# Autodesk Inventor assembly: ASY PNS 00 Panaevsk VOS
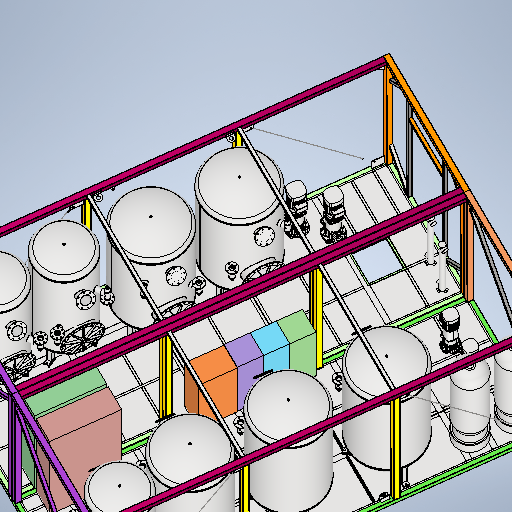
[picture p0: Inventor's stored thumbnail of the model, 512x512]
Saved by Autodesk Inventor 2025 (Build 290162010, 162A)
## iProperties
Created: 2025-02-24
Part Number: ASY PNS 00 Panaevsk VOS
Document SubType Name: Assembly
Designer: user
Author: user
## Documents named in this file (19)
- C:\Users\admin\Desktop\PNS-Panaevsk\ASY PNS 00 Panaevsk VOS.iam
- C:\Users\admin\Desktop\PNS-Panaevsk\Filter D1200\ASY PNS-Filter column D1200.iam
- C:\Users\admin\Desktop\PNS-Panaevsk\Filter D1000\ASY PNS-Filter column D1000.iam
- C:\Users\admin\Desktop\PNS-Panaevsk\ASY PNS-0100 MAIN FRAME.iam
- C:\Users\admin\Desktop\PNS-Panaevsk\ASY PNS-0200 FRAME 2.ipt
- C:\Users\admin\Desktop\PNS-Panaevsk\PNS-0921 concrete plate.ipt
- C:\Users\admin\Desktop\PNS-Panaevsk\PNS-0931 Sandwich wall.ipt
- C:\Users\admin\Desktop\PNS-Panaevsk\PNS-0932 Sandwich wall roof.ipt
- C:\Users\admin\Desktop\PNS-Panaevsk\PNS-0264 roof beam.ipt
- C:\Users\admin\Desktop\PNS-Panaevsk\Оборудование Инвентор\Вертикальный насос\CDM(F)15-4 FSWP(S_L)C\CDM(F)15-4 FSWP(S_L)C.iam
- C:\Users\admin\Desktop\PNS-Panaevsk\Оборудование Инвентор\Вертикальный насос\CDM(F)65-2-2 FSWP(S)C\CDM(F)65-2-2 FSWP(S)C.iam
- C:\Users\admin\Desktop\PNS-Panaevsk\Оборудование Инвентор\HY-H H2162–4T.ipt
- C:\Users\admin\Desktop\PNS-Panaevsk\Оборудование Инвентор\UV-Cleaner ODV-15.ipt
- C:\Users\admin\Desktop\PNS-Panaevsk\Оборудование Инвентор\Шкафы управления\Control box №1.ipt
- C:\Users\admin\Desktop\PNS-Panaevsk\Оборудование Инвентор\Шкафы управления\Control box №2.ipt
- C:\Users\admin\Desktop\PNS-Panaevsk\Оборудование Инвентор\Станции дозирования\Coagulant barrel.ipt
- C:\Users\admin\Desktop\PNS-Panaevsk\Оборудование Инвентор\Станции дозирования\Flocculant barrel.ipt
- C:\Users\admin\Desktop\PNS-Panaevsk\Оборудование Инвентор\Станции дозирования\GPHN barrel.ipt
- C:\Users\admin\Desktop\PNS-Panaevsk\Оборудование Инвентор\Станции дозирования\Soda barrel.ipt
## Components (34 placed, 18 different names)
1. ASY PNS-Filter column D1200:2 [sub-assembly] — Rigid:13
2. ASY PNS-Filter column D1000:3 [sub-assembly] — Rigid:16
3. ASY PNS-Filter column D1000:5 [sub-assembly] — Rigid:18
4. ASY PNS-0100 MAIN FRAME:1 [sub-assembly] — Rigid:1, Rigid:3, Rigid:4, Rigid:5, Rigid:7, Rigid:8, Rigid:9, Rigid:12, Rigid:13, Mate:15, Mate:16, Mate:17, Mate:18, Mate:19, Mate:20, Mate:21, Mate:22, Mate:23, Mate:24, Mate:26, Mate:27, Rigid:16, Rigid:17, Rigid:18
5. ASY PNS-0200 FRAME 2:1
6. ASY PNS-Filter column D1200:5 [sub-assembly] — Rigid:12
7. ASY PNS-Filter column D1200:6 [sub-assembly] — Rigid:8
8. ASY PNS-Filter column D1200:7 [sub-assembly] — Rigid:9
9. PNS-0931 Sandwich wall:1 — Rigid:1
10. PNS-0932 Sandwich wall roof:1 — Rigid:2
11. PNS-0932 Sandwich wall roof:2 — Rigid:2
12. PNS-0264 roof beam:1 — Rigid:3
13. PNS-0264 roof beam:2 — Rigid:4
14. PNS-0264 roof beam:3 — Rigid:5
15. ASY PNS-Filter column D1200:8 [sub-assembly] — Rigid:7
16. ASY PNS-Filter column D1000:6 [sub-assembly] — Rigid:17
17. CDM(F)15-4 FSWP(S_L)C:1 [sub-assembly] — Mate:16
18. CDM(F)65-2-2 FSWP(S)C:1 [sub-assembly] — Mate:18
19. HY-H H2162–4T:1 — Mate:19
20. UV-Cleaner ODV-15:1 — Mate:22
21. UV-Cleaner ODV-15:2 — Mate:21
22. HY-H H2162–4T:2 — Mate:20
23. CDM(F)65-2-2 FSWP(S)C:2 [sub-assembly] — Mate:17
24. CDM(F)15-4 FSWP(S_L)C:2 [sub-assembly] — Mate:15
25. Control box №1:1 — Mate:23, Mate:25, Flush:8
26. Control box №2:1 — Mate:24, Mate:25, Flush:8
27. Coagulant barrel:1 — Rigid:14, Rigid:15
28. Flocculant barrel:1 — Rigid:15, Mate:26
29. GPHN barrel:1 — Mate:27
30. Soda barrel:1 — Rigid:14
31. PNS-0921 concrete plate:1 — Flush:6, Flush:7, Mate:14
32. PNS-0921 concrete plate:2
33. PNS-0921 concrete plate:3
34. PNS-0921 concrete plate:4
## Component patterns: (4 elements, first: PNS-0921 concrete plate:1)
## Relationships (32: WeldJoint 15, Mate 14, Flush 3)
- Flush:6: PNS-0921 concrete plate:1
- Flush:7: PNS-0921 concrete plate:1
- Mate:14 (-500 mm): PNS-0921 concrete plate:1
- Rigid:1 [WeldJoint]: ASY PNS-0100 MAIN FRAME:1 ↔ PNS-0931 Sandwich wall:1
- Rigid:2 [WeldJoint]: PNS-0932 Sandwich wall roof:1 ↔ PNS-0932 Sandwich wall roof:2
- Rigid:3 [WeldJoint]: ASY PNS-0100 MAIN FRAME:1 ↔ PNS-0264 roof beam:1
- Rigid:4 [WeldJoint]: ASY PNS-0100 MAIN FRAME:1 ↔ PNS-0264 roof beam:2
- Rigid:5 [WeldJoint]: ASY PNS-0100 MAIN FRAME:1 ↔ PNS-0264 roof beam:3
- Rigid:7 [WeldJoint] (40 mm): ASY PNS-0100 MAIN FRAME:1 ↔ ASY PNS-Filter column D1200:8
- Rigid:8 [WeldJoint] (40 mm): ASY PNS-0100 MAIN FRAME:1 ↔ ASY PNS-Filter column D1200:6
- Rigid:9 [WeldJoint] (40 mm): ASY PNS-0100 MAIN FRAME:1 ↔ ASY PNS-Filter column D1200:7
- Rigid:12 [WeldJoint] (40 mm): ASY PNS-0100 MAIN FRAME:1 ↔ ASY PNS-Filter column D1200:5
- Rigid:13 [WeldJoint] (40 mm): ASY PNS-Filter column D1200:2 ↔ ASY PNS-0100 MAIN FRAME:1
- Mate:15: ASY PNS-0100 MAIN FRAME:1 ↔ CDM(F)15-4 FSWP(S_L)C:2
- Mate:16: ASY PNS-0100 MAIN FRAME:1 ↔ CDM(F)15-4 FSWP(S_L)C:1
- Mate:17: ASY PNS-0100 MAIN FRAME:1 ↔ CDM(F)65-2-2 FSWP(S)C:2
- Mate:18: ASY PNS-0100 MAIN FRAME:1 ↔ CDM(F)65-2-2 FSWP(S)C:1
- Mate:19: ASY PNS-0100 MAIN FRAME:1 ↔ HY-H H2162–4T:1
- Mate:20: ASY PNS-0100 MAIN FRAME:1 ↔ HY-H H2162–4T:2
- Mate:21: ASY PNS-0100 MAIN FRAME:1 ↔ UV-Cleaner ODV-15:2
- Mate:22: ASY PNS-0100 MAIN FRAME:1 ↔ UV-Cleaner ODV-15:1
- Mate:23: ASY PNS-0100 MAIN FRAME:1 ↔ Control box №1:1
- Mate:24: ASY PNS-0100 MAIN FRAME:1 ↔ Control box №2:1
- Mate:25 (50 mm): Control box №1:1 ↔ Control box №2:1
- Flush:8: Control box №1:1 ↔ Control box №2:1
- Rigid:14 [WeldJoint]: Coagulant barrel:1 ↔ Soda barrel:1
- Rigid:15 [WeldJoint]: Coagulant barrel:1 ↔ Flocculant barrel:1
- Mate:26: ASY PNS-0100 MAIN FRAME:1 ↔ Flocculant barrel:1
- Mate:27: ASY PNS-0100 MAIN FRAME:1 ↔ GPHN barrel:1
- Rigid:16 [WeldJoint] (40 mm): ASY PNS-Filter column D1000:3 ↔ ASY PNS-0100 MAIN FRAME:1
- Rigid:17 [WeldJoint] (40 mm): ASY PNS-0100 MAIN FRAME:1 ↔ ASY PNS-Filter column D1000:6
- Rigid:18 [WeldJoint] (40 mm): ASY PNS-Filter column D1000:5 ↔ ASY PNS-0100 MAIN FRAME:1
